# Autodesk Inventor assembly: holder_assembly
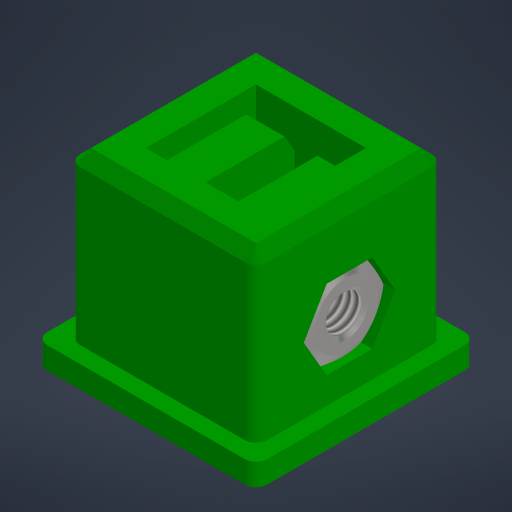
[picture p0: Inventor's stored thumbnail of the model, 512x512]
Saved by Autodesk Inventor 2024 (Build 280153000, 153)
## iProperties
Created: 2023-05-14
Part Number: holder_assembly
Document SubType Name: Assembly
Designer: user
Author: user
## Documents named in this file (3)
- D:\Docs\Robot\3d\motor_assembly\holder_assembly.iam
- D:\Docs\Robot\3d\motor_assembly\holder_assembly\holder.ipt
- C:\Users\user\Documents\Inventor\Content Center Files\R2024\ru-RU\DIN 934\DIN 934 - M4 x 0,7.ipt
## Components (3 placed, 2 different names)
1. holder:1 — Совмещение:1, Совмещение:2, Совмещение:3, Вставка:1, Вставка:2
2. DIN 934 - заменено на DIN EN 24032/28673/28674 M4:1 — Вставка:1
3. DIN 934 - заменено на DIN EN 24032/28673/28674 M4:2 — Вставка:2
## Relationships (5: Mate 3, Insert 2)
- Совмещение:1 [Mate]: holder:1
- Совмещение:2 [Mate]: holder:1
- Совмещение:3 [Mate]: holder:1
- Вставка:1 [Insert]: holder:1 ↔ DIN 934 - заменено на DIN EN 24032/28673/28674 M4:1
- Вставка:2 [Insert]: holder:1 ↔ DIN 934 - заменено на DIN EN 24032/28673/28674 M4:2
